# Autodesk Inventor assembly: Rail_Assembly
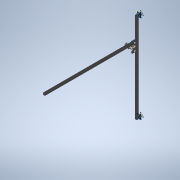
[picture p0: Inventor's stored thumbnail of the model, 180x180]
Saved by Autodesk Inventor 2021 (Build 250183000, 183)
## iProperties
Created: 2021-01-25
Part Number: Rail_Assembly
Document SubType Name: Assembly
Designer: Jorian Brusind
Mass: 3786.54 g
Surface Area: 19508.5 cm^2
Volume: 2323.9 cm^3
Density: 1.62939 g/cm^3
Author: Jorian Brusind
## Documents named in this file (18)
- C:\Users\Jorian Brusind\Documents\GitHub\PersonalProjects\HyperRail\Inventor Files\Rail_Assembly.iam
- C:\Users\Jorian Brusind\Documents\GitHub\PersonalProjects\Inventor Projects\Useful models\NEMA_Steppers\NEMA23\23HS8430B.ipt
- C:\Users\Jorian Brusind\Documents\GitHub\PersonalProjects\HyperRail\Inventor Files\NEMA23_StepperonlineMount.ipt
- C:\Users\Jorian Brusind\Documents\GitHub\PersonalProjects\HyperRail\Inventor Files\Roller_Bracket.iam
- C:\Users\Jorian Brusind\Documents\GitHub\PersonalProjects\Inventor Projects\Useful models\8020_Sets\IPT_20_Series\IPT_20_Series\20-2040_200mm.ipt
- C:\Users\Jorian Brusind\Documents\GitHub\PersonalProjects\HyperRail\Inventor Files\2804S_NEMA2115_1Gearbox.ipt
- C:\Users\Jorian Brusind\Documents\GitHub\PersonalProjects\Inventor Projects\Useful models\8020_Sets\IPT_40_Series\Extra_40_Series\90deg_4040.ipt
- C:\Users\Jorian Brusind\Documents\GitHub\PersonalProjects\HyperRail\Inventor Files\Bottom_Stand.ipt
- C:\Users\Jorian Brusind\Documents\GitHub\PersonalProjects\HyperRail\Inventor Files\SmallBelt_LargePulley.ipt
- C:\Users\Jorian Brusind\Documents\GitHub\PersonalProjects\HyperRail\Inventor Files\11mm_BearingWheel.ipt
- C:\Users\Jorian Brusind\Documents\GitHub\PersonalProjects\Inventor Projects\Useful models\Metric bolt\Bolt M5 25mm.ipt
- C:\Users\Jorian Brusind\Documents\GitHub\PersonalProjects\HyperRail\Inventor Files\Idlepulley_Spacer.ipt
- C:\Users\Jorian Brusind\Documents\GitHub\PersonalProjects\HyperRail\Inventor Files\Small_belt_5mm_1mm.ipt
- C:\Users\Jorian Brusind\Documents\GitHub\PersonalProjects\Inventor Projects\Useful models\8020_Sets\IPT_20_Series\Extra_20_Series\8020_14056m\14056_m.ipt
- C:\Users\Jorian Brusind\Documents\GitHub\PersonalProjects\HyperRail\PCB Files\Integrated Stepper Motor Driver\ExportSTEP\Main.iam
- C:\Users\Jorian Brusind\Documents\GitHub\PersonalProjects\HyperRail\Inventor Files\NEMA23_Shroud.ipt
- C:\Users\Jorian Brusind\Documents\GitHub\PersonalProjects\HyperRail\Inventor Files\NEMA23_Shroud_Cover.ipt
- C:\Users\Jorian Brusind\Documents\GitHub\PersonalProjects\Inventor Projects\Useful models\8020_Sets\IPT_20_Series\IPT_20_Series\20-4040_2m.ipt
## Components (25 placed, 17 different names)
1. 23HS8430B:1 — Angle:1, Mate:97, Mate:125, Flush:54, Flush:55, Mate:127, Mate:129, Mate:130, Mate:156
2. NEMA23_StepperonlineMount:1 — Angle:1, Angle:2, Mate:98, Mate:101, Mate:104, Mate:106, Mate:128, Mate:149, Mate:155, Flush:65
3. Roller_Bracket:1 [sub-assembly] — Flush:45, Mate:113, Mate:117, Flush:50, Mate:120, Flush:51, Mate:141, Flush:57
4. Roller_Bracket:2 [sub-assembly] — Flush:57, Mate:142, Flush:58, Mate:143, Mate:144, Mate:145
5. 20-2040_200mm:1 — Flush:34, Mate:83, Flush:35, Flush:36, Mate:85, Flush:45, Mate:113, Mate:118, Mate:119, Mate:121, Mate:124, Flush:56, Mate:142, Flush:58, Flush:59, Flush:60, Flush:63, Mate:151
6. 2804S_NEMA2115_1Gearbox:1 — Angle:2, Mate:97, Mate:98, Mate:99, Mate:100, Mate:109, Mate:127, Mate:128
7. 90deg_4040:1 — Flush:34, Mate:83, Flush:35, Mate:150
8. 90deg_4040:2 — Flush:36, Mate:85, Mate:149, Mate:152
9. Bottom_Stand:1 — Mate:136, Mate:137, Mate:138
10. Bottom_Stand:2 — Mate:133, Mate:134, Mate:135
11. SmallBelt_LargePulley:1 — Mate:99, Mate:100
12. 11mm_BearingWheel:1 — Mate:101, Mate:102, Mate:103, Mate:104
13. Bolt M5 25mm:1 — Mate:102, Mate:103, Mate:105
14. Idlepulley_Spacer:1 — Mate:105, Mate:106
15. Small_belt_5mm_1mm:1 — Mate:109, Flush:42, Mate:111, Flush:64
16. Small_belt_5mm_1mm:2 — Flush:42, Mate:111, Mate:153, Mate:154, Flush:64
17. 14056_m:1 — Mate:117, Mate:118, Flush:50
18. 14056_m:2 — Mate:119, Mate:120, Flush:51
19. 14056_m:3 — Mate:121, Mate:144, Flush:60
20. 14056_m:4 — Mate:124, Mate:143, Flush:59
21. Main:1 [sub-assembly] — Mate:125, Flush:54, Flush:55
22. NEMA23_Shroud:1 — Mate:129, Mate:130, Mate:131, Mate:132, Mate:156, Mate:157
23. NEMA23_Shroud_Cover:1 — Mate:131, Mate:132, Mate:157
24. 20-4040_2m:1 — Mate:133, Mate:134, Mate:135, Mate:136, Mate:137, Mate:138, Mate:139, Mate:140, Mate:141, Flush:56, Mate:145, Mate:153, Mate:154
25. 20-4040_2m:2 — Mate:150, Flush:63, Mate:151, Mate:152, Mate:155, Flush:65
## Relationships (69: Mate 50, Flush 17, Angle 2)
- Angle:1 (0 deg): 23HS8430B:1 ↔ NEMA23_StepperonlineMount:1
- Angle:2 (0 deg): NEMA23_StepperonlineMount:1 ↔ 2804S_NEMA2115_1Gearbox:1
- Flush:34: 20-2040_200mm:1 ↔ 90deg_4040:1
- Mate:83: 20-2040_200mm:1 ↔ 90deg_4040:1
- Flush:35: 20-2040_200mm:1 ↔ 90deg_4040:1
- Flush:36: 20-2040_200mm:1 ↔ 90deg_4040:2
- Mate:85: 20-2040_200mm:1 ↔ 90deg_4040:2
- Mate:97: 23HS8430B:1 ↔ 2804S_NEMA2115_1Gearbox:1
- Mate:98: NEMA23_StepperonlineMount:1 ↔ 2804S_NEMA2115_1Gearbox:1
- Mate:99: 2804S_NEMA2115_1Gearbox:1 ↔ SmallBelt_LargePulley:1
- Mate:100 (4 mm): 2804S_NEMA2115_1Gearbox:1 ↔ SmallBelt_LargePulley:1
- Mate:101: NEMA23_StepperonlineMount:1 ↔ 11mm_BearingWheel:1
- Mate:102: 11mm_BearingWheel:1 ↔ Bolt M5 25mm:1
- Mate:103: 11mm_BearingWheel:1 ↔ Bolt M5 25mm:1
- Mate:104 (10 mm): NEMA23_StepperonlineMount:1 ↔ 11mm_BearingWheel:1
- Mate:105: Bolt M5 25mm:1 ↔ Idlepulley_Spacer:1
- Mate:106: NEMA23_StepperonlineMount:1 ↔ Idlepulley_Spacer:1
- Mate:109 (10 mm): 2804S_NEMA2115_1Gearbox:1 ↔ Small_belt_5mm_1mm:1
- Flush:42: Small_belt_5mm_1mm:1 ↔ Small_belt_5mm_1mm:2
- Mate:111 (20 mm): Small_belt_5mm_1mm:1 ↔ Small_belt_5mm_1mm:2
- Flush:45: Roller_Bracket:1 ↔ 20-2040_200mm:1
- Mate:113: Roller_Bracket:1 ↔ 20-2040_200mm:1
- Mate:117: Roller_Bracket:1 ↔ 14056_m:1
- Mate:118: 20-2040_200mm:1 ↔ 14056_m:1
- Flush:50: Roller_Bracket:1 ↔ 14056_m:1
- Mate:119: 20-2040_200mm:1 ↔ 14056_m:2
- Mate:120: Roller_Bracket:1 ↔ 14056_m:2
- Flush:51: Roller_Bracket:1 ↔ 14056_m:2
- Mate:121: 20-2040_200mm:1 ↔ 14056_m:3
- Mate:124: 20-2040_200mm:1 ↔ 14056_m:4
- Mate:125 (1 mm): 23HS8430B:1 ↔ Main:1
- Flush:54 (7 mm): 23HS8430B:1 ↔ Main:1
- Flush:55 (7 mm): 23HS8430B:1 ↔ Main:1
- Mate:127: 23HS8430B:1 ↔ 2804S_NEMA2115_1Gearbox:1
- Mate:128: NEMA23_StepperonlineMount:1 ↔ 2804S_NEMA2115_1Gearbox:1
- Mate:129: 23HS8430B:1 ↔ NEMA23_Shroud:1
- Mate:130: 23HS8430B:1 ↔ NEMA23_Shroud:1
- Mate:131: NEMA23_Shroud:1 ↔ NEMA23_Shroud_Cover:1
- Mate:132: NEMA23_Shroud:1 ↔ NEMA23_Shroud_Cover:1
- Mate:133: Bottom_Stand:2 ↔ 20-4040_2m:1
- Mate:134: Bottom_Stand:2 ↔ 20-4040_2m:1
- Mate:135: Bottom_Stand:2 ↔ 20-4040_2m:1
- Mate:136: Bottom_Stand:1 ↔ 20-4040_2m:1
- Mate:137: Bottom_Stand:1 ↔ 20-4040_2m:1
- Mate:138: Bottom_Stand:1 ↔ 20-4040_2m:1
- Mate:139: 20-4040_2m:1
- Mate:140: 20-4040_2m:1
- Mate:141 (11 mm): Roller_Bracket:1 ↔ 20-4040_2m:1
- Flush:56: 20-2040_200mm:1 ↔ 20-4040_2m:1
- Flush:57: Roller_Bracket:1 ↔ Roller_Bracket:2
- Mate:142: Roller_Bracket:2 ↔ 20-2040_200mm:1
- Flush:58: Roller_Bracket:2 ↔ 20-2040_200mm:1
- Mate:143: Roller_Bracket:2 ↔ 14056_m:4
- Flush:59: 20-2040_200mm:1 ↔ 14056_m:4
- Mate:144: Roller_Bracket:2 ↔ 14056_m:3
- Flush:60: 20-2040_200mm:1 ↔ 14056_m:3
- Mate:145 (1 mm): Roller_Bracket:2 ↔ 20-4040_2m:1
- Mate:149: NEMA23_StepperonlineMount:1 ↔ 90deg_4040:2
- Mate:150: 90deg_4040:1 ↔ 20-4040_2m:2
- Flush:63: 20-2040_200mm:1 ↔ 20-4040_2m:2
- Mate:151: 20-2040_200mm:1 ↔ 20-4040_2m:2
- Mate:152: 90deg_4040:2 ↔ 20-4040_2m:2
- Mate:153: Small_belt_5mm_1mm:2 ↔ 20-4040_2m:1
- Mate:154: Small_belt_5mm_1mm:2 ↔ 20-4040_2m:1
- Flush:64: Small_belt_5mm_1mm:1 ↔ Small_belt_5mm_1mm:2
- Mate:155: NEMA23_StepperonlineMount:1 ↔ 20-4040_2m:2
- Flush:65: NEMA23_StepperonlineMount:1 ↔ 20-4040_2m:2
- Mate:156: 23HS8430B:1 ↔ NEMA23_Shroud:1
- Mate:157: NEMA23_Shroud:1 ↔ NEMA23_Shroud_Cover:1
